# Autodesk Inventor assembly: Assembly2
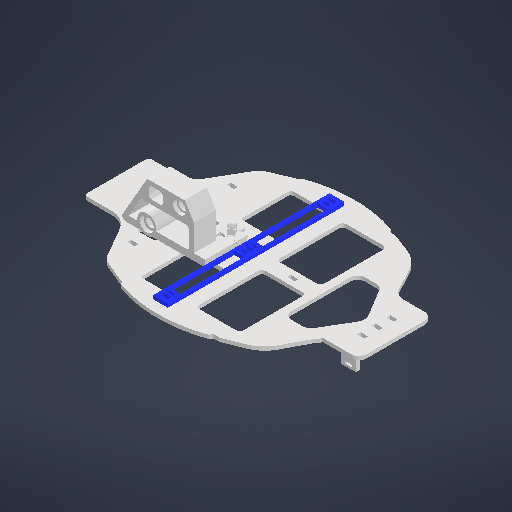
[picture p0: Inventor's stored thumbnail of the model, 512x512]
Saved by Autodesk Inventor 2025.3 (Build 293356000, 356)
## iProperties
Created: 2025-11-13
Part Number: Assembly2
Document SubType Name: Assembly
Designer: sophi
Author: sophi
## Documents named in this file (5)
- C:\Users\sophi\OneDrive - Universidad de los andes\Documentos\1 Universidad\5 Semestre\Proyecto\Huron-Hudson\Pelton Engine\V12\Assembly2.iam
- C:\Users\sophi\OneDrive - Universidad de los andes\Documentos\1 Universidad\5 Semestre\Proyecto\Huron-Hudson\Pelton Engine\V12\base botellas.ipt
- C:\Users\sophi\OneDrive - Universidad de los andes\Documentos\1 Universidad\5 Semestre\Proyecto\Huron-Hudson\Pelton Engine\V12\base.ipt
- C:\Users\sophi\OneDrive - Universidad de los andes\Documentos\1 Universidad\5 Semestre\Proyecto\Huron-Hudson\Pelton Engine\V12\fixer.ipt
- C:\Users\sophi\OneDrive - Universidad de los andes\Documentos\1 Universidad\5 Semestre\Proyecto\Huron-Hudson\Pelton Engine\V12\Base Final.ipt
## Components (4 placed, 4 different names)
1. base botellas:1 — Mate:6, Flush:2, Flush:3
2. base:1 — Mate:3, Mate:5
3. fixer:1 — Mate:3
4. Base Final:1 — Mate:1, Flush:1, Mate:2, Mate:5, Mate:6, Flush:2, Flush:3
## Relationships (8: Mate 5, Flush 3)
- Mate:1: Base Final:1
- Flush:1: Base Final:1
- Mate:2: Base Final:1
- Mate:3: base:1 ↔ fixer:1
- Mate:5: base:1 ↔ Base Final:1
- Mate:6: base botellas:1 ↔ Base Final:1
- Flush:2: base botellas:1 ↔ Base Final:1
- Flush:3: base botellas:1 ↔ Base Final:1
